# Autodesk Inventor assembly: czlon i przekladnia
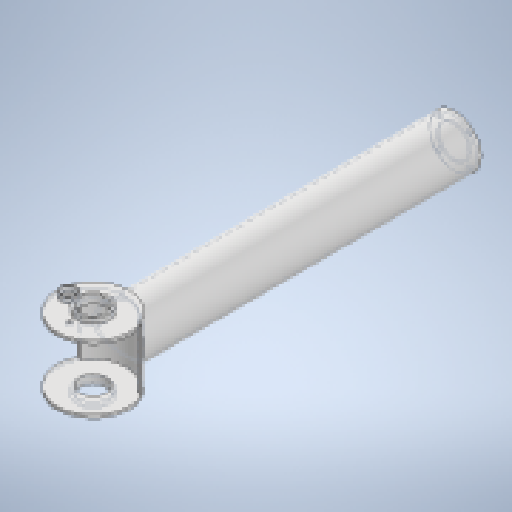
[picture p0: Inventor's stored thumbnail of the model, 512x512]
Saved by Autodesk Inventor 2023 (Build 270158000, 158)
## iProperties
Created: 2023-04-08
Part Number: czlon i przekladnia
Document SubType Name: Assembly
Designer: Wiktor
Author: Wiktor
## Documents named in this file (2)
- C:\Users\krzys\Documents\GitHub\Manipulator-Inventor\czlon i przekladnia.iam
- C:\Users\krzys\Documents\GitHub\Manipulator-Inventor\czlon_1.ipt
## Components (1 placed, 1 different names)
1. czlon_1:1 — Zestawiające:7
## Relationships (2: Mate 2)
- Zestawiające:7 [Mate]: czlon_1:1
- Zestawiające:8 [Mate]
